# Autodesk Inventor assembly: Actuador
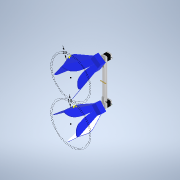
[picture p0: Inventor's stored thumbnail of the model, 180x180]
Saved by Autodesk Inventor 2022 (Build 260153000, 153)
## iProperties
Created: 2023-10-27
Part Number: Actuador
Document SubType Name: Assembly
Designer: jp.reyesf
Author: jp.reyesf
## Documents named in this file (6)
- C:\Users\jp.reyesf\Documents\GPR Portable\Actuador\Actuador.iam
- C:\Users\jp.reyesf\Documents\GPR Portable\Antenas\Antena PowerLog.ipt
- C:\Users\jp.reyesf\Documents\GPR Portable\Motores\M1173041- NEMA 17.ipt
- C:\Users\jp.reyesf\Documents\GPR Portable\Motores\Acople Motor.ipt
- C:\Users\jp.reyesf\Documents\GPR Portable\Estructura\Soporte motores actuador.ipt
- C:\Users\jp.reyesf\Documents\GPR Portable\Estructura\VSLOT 2020 actuador.ipt
## Components (8 placed, 5 different names)
1. Antena PowerLog:1 — Coincidencia:1, Nivelación:1, Nivelación:2, Tangente:1
2. M1173041- NEMA 17:1 — Coincidencia:1, Coincidencia:2, Nivelación:3, Nivelación:4, Nivelación:7, Nivelación:8, Coincidencia:7
3. Acople Motor:1 — Nivelación:1, Nivelación:2, Coincidencia:2
4. Soporte motores actuador:1 — Nivelación:3, Nivelación:4, Coincidencia:6, Nivelación:9
5. Antena PowerLog:2 — Tangente:1
6. M1173041- NEMA 17:2 — Coincidencia:5, Nivelación:7, Nivelación:8
7. Acople Motor:2 — Coincidencia:5
8. VSLOT 2020 actuador:1 — Coincidencia:6, Nivelación:9, Coincidencia:7
## Relationships (17: Flush 9, Mate 7, Tangent 1)
- Coincidencia:1 [Mate]: Antena PowerLog:1 ↔ M1173041- NEMA 17:1
- Nivelación:1 [Flush]: Antena PowerLog:1 ↔ Acople Motor:1
- Nivelación:2 [Flush]: Antena PowerLog:1 ↔ Acople Motor:1
- Coincidencia:2 [Mate]: M1173041- NEMA 17:1 ↔ Acople Motor:1
- Nivelación:3 [Flush]: M1173041- NEMA 17:1 ↔ Soporte motores actuador:1
- Nivelación:4 [Flush]: M1173041- NEMA 17:1 ↔ Soporte motores actuador:1
- [Mate]: Antena PowerLog:2 ↔ M1173041- NEMA 17:2
- [Flush]: Antena PowerLog:2 ↔ Acople Motor:2
- [Flush]: Antena PowerLog:2 ↔ Acople Motor:2
- [Mate]: M1173041- NEMA 17:2 ↔ Acople Motor:2
- Coincidencia:5 [Mate]: M1173041- NEMA 17:2 ↔ Acople Motor:2
- Nivelación:7 [Flush]: M1173041- NEMA 17:1 ↔ M1173041- NEMA 17:2
- Nivelación:8 [Flush]: M1173041- NEMA 17:1 ↔ M1173041- NEMA 17:2
- Tangente:1: Antena PowerLog:1 ↔ Antena PowerLog:2
- Coincidencia:6 [Mate]: Soporte motores actuador:1 ↔ VSLOT 2020 actuador:1
- Nivelación:9 [Flush]: Soporte motores actuador:1 ↔ VSLOT 2020 actuador:1
- Coincidencia:7 [Mate]: M1173041- NEMA 17:1 ↔ VSLOT 2020 actuador:1
## Named parameters: d7_d3 = 0 mm, d8_d4 = 0 mm, d9_d0 = 0 mm, d10_d2 = 0 mm
